# Autodesk Inventor assembly: Pump Set
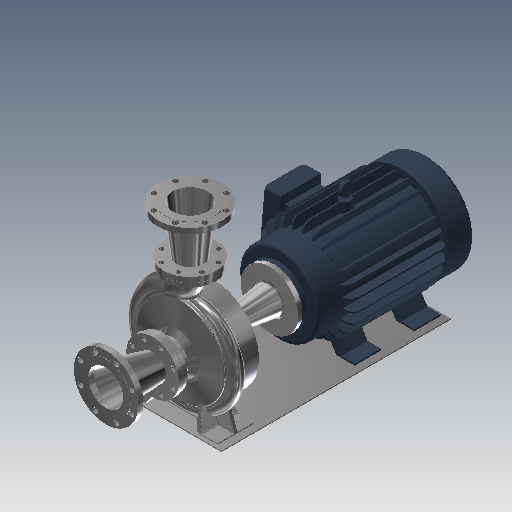
[picture p0: Inventor's stored thumbnail of the model, 512x512]
Saved by Autodesk Inventor 2020 (Build 240152000, 152)
## iProperties
Created: 2018-09-07
Part Number: Pump Set
Document SubType Name: Assembly
Designer: alid
Author: alid
## Documents named in this file (5)
- C:\Users\hallc\Desktop\Process Equipment\Workspace\Options\Pump Set.iam
- C:\Users\hallc\Desktop\Process Equipment\Workspace\Options\Centrifugal Pump.ipt
- C:\Users\hallc\Desktop\Process Equipment\Workspace\Components\ASME B16.5 Flanged Reducer - Class 150 6 x 4 St Stl.ipt
- C:\Users\hallc\Desktop\Process Equipment\Workspace\Components\ASME B16.5 Flanged Eccentric Reducer - Class 150 6 x 4 St Stl.ipt
- C:\Users\hallc\Desktop\Process Equipment\Workspace\Components\Pump Set Skid Plate.ipt
## Components (4 placed, 4 different names)
1. Pump Set Skid Plate:1 — Mate:1, Mate:2, Flush:1
2. Centrifugal Pump:1 — Rigid:1, Rigid:2, Mate:1, Mate:2, Flush:1
3. ASME B16.5 Flanged Eccentric Reducer - Class 150 6 x 4 St Stl:1 — Rigid:1
4. ASME B16.5 Flanged Reducer - Class 150 6 x 4 St Stl:1 — Rigid:2
## Relationships (5: WeldJoint 2, Mate 2, Flush 1)
- Rigid:1 [WeldJoint]: Centrifugal Pump:1 ↔ ASME B16.5 Flanged Eccentric Reducer - Class 150 6 x 4 St Stl:1
- Rigid:2 [WeldJoint]: Centrifugal Pump:1 ↔ ASME B16.5 Flanged Reducer - Class 150 6 x 4 St Stl:1
- Mate:1: Pump Set Skid Plate:1 ↔ Centrifugal Pump:1
- Mate:2: Pump Set Skid Plate:1 ↔ Centrifugal Pump:1
- Flush:1 (15 mm): Pump Set Skid Plate:1 ↔ Centrifugal Pump:1
